# Autodesk Inventor assembly: Y linear rail mounts assebly for milling
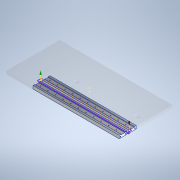
[picture p0: Inventor's stored thumbnail of the model, 180x180]
Saved by Autodesk Inventor 2020 (Build 240168000, 168)
## iProperties
Created: 2019-05-20
Part Number: Y linear rail mounts assebly for milling
Document SubType Name: Assembly
Designer: LillaHunden
Author: LillaHunden
## Documents named in this file (3)
- C:\Users\LillaHunden\Documents\Inventor\3dprinter\3dPrinter\Y linear rail mounts assebly for milling.iam
- C:\Users\LillaHunden\Documents\Inventor\3dprinter\3dPrinter\rails stock solid.ipt
- C:\Users\LillaHunden\Documents\Inventor\3dprinter\3dPrinter\Frame Bottom Front.ipt
## Components (3 placed, 2 different names)
1. rails stock solid:1 — Flush:3, Flush:4, Flush:6
2. Frame Bottom Front:1 — Flush:1, Mate:1, Flush:2, Flush:4, Flush:5, Flush:6
3. Frame Bottom Front:2 — Flush:1, Mate:1, Flush:2, Flush:3, Flush:5
## Relationships (7: Flush 6, Mate 1)
- Flush:1: Frame Bottom Front:1 ↔ Frame Bottom Front:2
- Mate:1 (6 mm): Frame Bottom Front:1 ↔ Frame Bottom Front:2
- Flush:2: Frame Bottom Front:1 ↔ Frame Bottom Front:2
- Flush:3 (2 mm): rails stock solid:1 ↔ Frame Bottom Front:2
- Flush:4: rails stock solid:1 ↔ Frame Bottom Front:1
- Flush:5: Frame Bottom Front:1 ↔ Frame Bottom Front:2
- Flush:6 (86 mm): rails stock solid:1 ↔ Frame Bottom Front:1
